# Autodesk Inventor assembly: postStandSupport
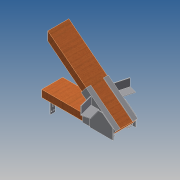
[picture p0: Inventor's stored thumbnail of the model, 180x180]
Saved by Autodesk Inventor 2014 SP1 (Build 180222100, 222)
## iProperties
Created: 2014-08-29
Part Number: postStandSupport
Document SubType Name: Assembly
Designer: Dave
Author: Dave
## Documents named in this file (6)
- C:\Users\Dave\Desktop\hera-cad\support\postStandSupport.iam
- C:\Users\Dave\Desktop\hera-cad\support\postStandHoriz.ipt
- C:\Users\Dave\Desktop\hera-cad\support\postStand37.ipt
- C:\Users\Dave\Desktop\hera-cad\smallParts\angleBracket.ipt
- C:\Users\Dave\Desktop\hera-cad\support\endcaps\HERA_end_cap_left.iam
- C:\Users\Dave\Desktop\hera-cad\support\endcaps\HERA_end_cap_right.iam
## Components (5 placed, 5 different names)
1. HERA_end_cap_left:1 [sub-assembly] — Mate:8, Mate:9, Flush:2, Mate:10, Mate:11, Flush:3, Flush:4, Flush:5
2. postStandHoriz:1 — Mate:7, Flush:1, Mate:8, Mate:9, Flush:2, Mate:12, Flush:6
3. postStand37:1 — Mate:10, Mate:11, Flush:3
4. angleBracket:1 — Mate:7, Flush:1, Flush:6
5. HERA_end_cap_right:1 [sub-assembly] — Mate:12, Flush:4, Flush:5
## Relationships (12: Mate 6, Flush 6)
- Mate:7: postStandHoriz:1 ↔ angleBracket:1
- Flush:1: postStandHoriz:1 ↔ angleBracket:1
- Mate:8: HERA_end_cap_left:1 ↔ postStandHoriz:1
- Mate:9: HERA_end_cap_left:1 ↔ postStandHoriz:1
- Flush:2 (-37 mm): HERA_end_cap_left:1 ↔ postStandHoriz:1
- Mate:10: HERA_end_cap_left:1 ↔ postStand37:1
- Mate:11: HERA_end_cap_left:1 ↔ postStand37:1
- Flush:3: HERA_end_cap_left:1 ↔ postStand37:1
- Mate:12: postStandHoriz:1 ↔ HERA_end_cap_right:1
- Flush:4: HERA_end_cap_left:1 ↔ HERA_end_cap_right:1
- Flush:5: HERA_end_cap_left:1 ↔ HERA_end_cap_right:1
- Flush:6 (-44.3 mm): postStandHoriz:1 ↔ angleBracket:1
